# Autodesk Inventor assembly: 155
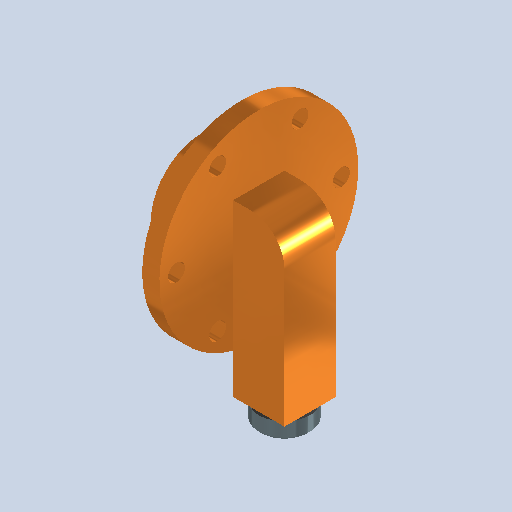
[picture p0: Inventor's stored thumbnail of the model, 512x512]
Saved by Autodesk Inventor 2025.1 (Build 291241000, 241)
## iProperties
Created: 2024-08-03
Part Number: 155
Document SubType Name: Assembly
Designer: ffogue
Author: ffogue
## Documents named in this file (3)
- C:\Projkete - Übungen\Freedom\155.iam
- C:\Projkete - Übungen\Freedom\155 part 1.ipt
- C:\Projkete - Übungen\Freedom\155 part 2.iam
## Components (2 placed, 2 different names)
1. 155 part 1:1 — Insert:1
2. 155 part 2:1 [sub-assembly] — Insert:1
## Relationships (1: Insert 1)
- Insert:1: 155 part 1:1 ↔ 155 part 2:1
